# Autodesk Inventor assembly: Assembly1
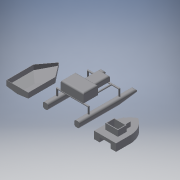
[picture p0: Inventor's stored thumbnail of the model, 180x180]
Saved by Autodesk Inventor 2016 (Build 200138000, 138)
## iProperties
Created: 2019-01-14
Part Number: Assembly1
Document SubType Name: Assembly
Designer: LinJie
Author: LinJie
## Documents named in this file (4)
- C:\Users\LinJie\Documents\Inventor\EA Water project\Assembly1.iam
- C:\Users\LinJie\Documents\Inventor\EA Water project\Generalcraftshape1.ipt
- C:\Users\LinJie\Documents\Inventor\EA Water project\GeneralCraftShape2.ipt
- C:\Users\LinJie\Documents\Inventor\EA Water project\GeneralCraftShape3.ipt
## Components (3 placed, 3 different names)
1. Generalcraftshape1:1 — Mate:1, Flush:1, Flush:2
2. GeneralCraftShape2:1 — Mate:1, Flush:1, Flush:2, Mate:2, Flush:3, Flush:4
3. GeneralCraftShape3:1 — Mate:2, Flush:3, Flush:4
## Relationships (6: Flush 4, Mate 2)
- Mate:1 (200 mm): Generalcraftshape1:1 ↔ GeneralCraftShape2:1
- Flush:1: Generalcraftshape1:1 ↔ GeneralCraftShape2:1
- Flush:2: Generalcraftshape1:1 ↔ GeneralCraftShape2:1
- Mate:2 (200 mm): GeneralCraftShape2:1 ↔ GeneralCraftShape3:1
- Flush:3: GeneralCraftShape2:1 ↔ GeneralCraftShape3:1
- Flush:4: GeneralCraftShape2:1 ↔ GeneralCraftShape3:1
